# Autodesk Inventor assembly: CNC-FullAssembly
(part 3 of 3)
- Mate:441: CNC-014-ZAxisSubMount1:1 ↔ 90327A125-M5x10mm-LowProfileSCS:17
- Mate:442: CNC-014-ZAxisSubMount1:1 ↔ 90327A125-M5x10mm-LowProfileSCS:18
- Flush:214: 90327A125-M5x10mm-LowProfileSCS:17 ↔ 90327A125-M5x10mm-LowProfileSCS:18
- Flush:215: 90327A125-M5x10mm-LowProfileSCS:13 ↔ 90327A125-M5x10mm-LowProfileSCS:17
- Mate:443: BF12-BallScrewStabilizer2:1 ↔ 91290A195-M5x35mm:2
- Mate:444: BF12-BallScrewStabilizer2:1 ↔ 91290A195-M5x35mm:4
- Mate:445: BF12-BallScrewStabilizer2:1 ↔ 91290A195-M5x35mm:1
- Mate:446: BF12-BallScrewStabilizer2:1 ↔ 91290A195-M5x35mm:3
- Mate:447: BF12-BallScrewStabilizer2:1 ↔ 91290A195-M5x35mm:3
- Flush:216: 91290A195-M5x35mm:2 ↔ 91290A195-M5x35mm:3
- Flush:217: 91290A195-M5x35mm:2 ↔ 91290A195-M5x35mm:4
- Flush:218: 91290A195-M5x35mm:1 ↔ 91290A195-M5x35mm:4
- Mate:448: 91290A195-M5x35mm:2 ↔ 90576A104-M5-NylockNut:9
- Mate:449: 91290A195-M5x35mm:3 ↔ 90576A104-M5-NylockNut:10
- Mate:450: 91290A195-M5x35mm:4 ↔ 90576A104-M5-NylockNut:11
- Mate:451: 91290A195-M5x35mm:1 ↔ 90576A104-M5-NylockNut:12
- Mate:452: CNC-001-StructureGusset2:1 ↔ 90576A104-M5-NylockNut:9
- Flush:219: 90576A104-M5-NylockNut:9 ↔ 90576A104-M5-NylockNut:10
- Flush:220: 90576A104-M5-NylockNut:10 ↔ 90576A104-M5-NylockNut:12
- Flush:221: 90576A104-M5-NylockNut:11 ↔ 90576A104-M5-NylockNut:12
- Mate:453: RouterSpindle-65mm:1 ↔ CNC-015-65mmSpindleMount:1
- Mate:454: RouterSpindle-65mm:1 ↔ CNC-015-65mmSpindleMount:1
- Mate:455: HGR20R-LinearRail200mm:2 ↔ 20x20x250mm_Extrusion:1
- Flush:222: HGR20R-LinearRail200mm:2 ↔ 20x20x250mm_Extrusion:1
- Flush:223: HGR20R-LinearRail200mm:2 ↔ 20x20x250mm_Extrusion:1
- Mate:456: HGR20R-LinearRail200mm:1 ↔ 20x20x250mm_Extrusion:2
- Flush:224: HGR20R-LinearRail200mm:1 ↔ 20x20x250mm_Extrusion:2
- Flush:225: 20x20x250mm_Extrusion:1 ↔ 20x20x250mm_Extrusion:2
- Mate:457: HGR20R-LinearRail200mm:2 ↔ 91290A231-M5x15mm:100
- Mate:458: HGR20R-LinearRail200mm:2 ↔ 91290A231-M5x15mm:100
- Mate:459: HGR20R-LinearRail200mm:1 ↔ 91290A231-M5x15mm:101
- Mate:460: HGR20R-LinearRail200mm:1 ↔ 91290A231-M5x15mm:102
- Mate:461: HGR20R-LinearRail200mm:1 ↔ 91290A231-M5x15mm:103
- Mate:462: HGR20R-LinearRail200mm:2 ↔ 91290A231-M5x15mm:104
- Mate:463: HGR20R-LinearRail200mm:2 ↔ 91290A231-M5x15mm:105
- Flush:226: 91290A231-M5x15mm:104 ↔ 91290A231-M5x15mm:105
- Flush:227: 91290A231-M5x15mm:100 ↔ 91290A231-M5x15mm:104
- Flush:228: 91290A231-M5x15mm:100 ↔ 91290A231-M5x15mm:101
- Flush:229: 91290A231-M5x15mm:101 ↔ 91290A231-M5x15mm:102
- Flush:230: 91290A231-M5x15mm:102 ↔ 91290A231-M5x15mm:103
- Mate:464: HGR20R-LinearRail200mm:1 ↔ 91290A231-M5x15mm:106
- Mate:465: HGR20R-LinearRail200mm:2 ↔ 91290A231-M5x15mm:107
- Flush:231: 91290A231-M5x15mm:100 ↔ 91290A231-M5x15mm:107
- Flush:232: 91290A231-M5x15mm:100 ↔ 91290A231-M5x15mm:106
- Angle:23 (0 deg): CNC-015-65mmSpindleMount:1 ↔ 20x20x250mm_Extrusion:1
- Mate:466: CNC-014-ZAxisSubMount1:1 ↔ 90327A125-M5x10mm-LowProfileSCS:19
- Mate:467: CNC-014-ZAxisSubMount1:1 ↔ 90327A125-M5x10mm-LowProfileSCS:20
- Flush:233: 90327A125-M5x10mm-LowProfileSCS:19 ↔ 90327A125-M5x10mm-LowProfileSCS:20
- Flush:234: 90327A125-M5x10mm-LowProfileSCS:16 ↔ 90327A125-M5x10mm-LowProfileSCS:19
- Mate:468: BF12-BallScrewStabilizer2:3 ↔ CNC-016-SpindleMountPlate:1
- Mate:469: BF12-BallScrewStabilizer2:3 ↔ CNC-016-SpindleMountPlate:1
- Mate:470: 20x20x250mm_Extrusion:2 ↔ CNC-016-SpindleMountPlate:1
- Mate:471: CNC-016-SpindleMountPlate:1 ↔ 90576A104-M5-NylockNut:13
- Mate:472: CNC-016-SpindleMountPlate:1 ↔ 90576A104-M5-NylockNut:13
- Mate:473: CNC-016-SpindleMountPlate:1 ↔ 90576A104-M5-NylockNut:14
- Flush:235: 90576A104-M5-NylockNut:13 ↔ 90576A104-M5-NylockNut:14
- Mate:474: CNC-016-SpindleMountPlate:1 ↔ 90576A104-M5-NylockNut:15
- Mate:475: CNC-016-SpindleMountPlate:1 ↔ 90576A104-M5-NylockNut:16
- Flush:236: 90576A104-M5-NylockNut:15 ↔ 90576A104-M5-NylockNut:16
- Flush:237: 90576A104-M5-NylockNut:13 ↔ 90576A104-M5-NylockNut:15
- Mate:476: CNC-015-65mmSpindleMount:1 ↔ 91274A131_M5x20mm:23
- Mate:477: CNC-015-65mmSpindleMount:1 ↔ 91274A131_M5x20mm:24
- Mate:478: CNC-015-65mmSpindleMount:1 ↔ 91274A131_M5x20mm:25
- Mate:479: CNC-015-65mmSpindleMount:1 ↔ 91274A131_M5x20mm:26
- Flush:238: 91274A131_M5x20mm:25 ↔ 91274A131_M5x20mm:26
- Flush:239: 91274A131_M5x20mm:23 ↔ 91274A131_M5x20mm:26
- Flush:240: 91274A131_M5x20mm:23 ↔ 91274A131_M5x20mm:24
- Mate:480: CNC-015-65mmSpindleMount:1 ↔ 91274A131_M5x20mm:23
- Mate:481: CNC-016-SpindleMountPlate:1 ↔ 90327A125-M5x10mm-LowProfileSCS:21
- Mate:482: CNC-016-SpindleMountPlate:1 ↔ 90327A125-M5x10mm-LowProfileSCS:21
- Mate:483: CNC-016-SpindleMountPlate:1 ↔ 90327A125-M5x10mm-LowProfileSCS:22
- Flush:241: 90327A125-M5x10mm-LowProfileSCS:21 ↔ 90327A125-M5x10mm-LowProfileSCS:22
- Mate:484: CNC-016-SpindleMountPlate:1 ↔ 90327A125-M5x10mm-LowProfileSCS:23
- Mate:485: CNC-016-SpindleMountPlate:1 ↔ 90327A125-M5x10mm-LowProfileSCS:24
- Flush:242: 90327A125-M5x10mm-LowProfileSCS:23 ↔ 90327A125-M5x10mm-LowProfileSCS:24
- Flush:243: 90327A125-M5x10mm-LowProfileSCS:22 ↔ 90327A125-M5x10mm-LowProfileSCS:23
- Mate:486: CNC-016-SpindleMountPlate:1 ↔ 90327A125-M5x10mm-LowProfileSCS:26
- Mate:487: CNC-016-SpindleMountPlate:1 ↔ 90327A125-M5x10mm-LowProfileSCS:27
- Mate:488: CNC-016-SpindleMountPlate:1 ↔ 90327A125-M5x10mm-LowProfileSCS:25
- Mate:489: CNC-016-SpindleMountPlate:1 ↔ 90327A125-M5x10mm-LowProfileSCS:28
- Flush:244: 90327A125-M5x10mm-LowProfileSCS:25 ↔ 90327A125-M5x10mm-LowProfileSCS:28
- Flush:245: 90327A125-M5x10mm-LowProfileSCS:27 ↔ 90327A125-M5x10mm-LowProfileSCS:28
- Flush:246: 90327A125-M5x10mm-LowProfileSCS:26 ↔ 90327A125-M5x10mm-LowProfileSCS:27
- Flush:247: 90327A125-M5x10mm-LowProfileSCS:21 ↔ 90327A125-M5x10mm-LowProfileSCS:26
- Mate:490: BK12-BallScrewStabilizer:3 ↔ 92981A790-M5x40mm-ShoulderBolt:5
- Mate:491: BK12-BallScrewStabilizer:3 ↔ 92981A790-M5x40mm-ShoulderBolt:3
- Mate:492: BK12-BallScrewStabilizer:3 ↔ 92981A790-M5x40mm-ShoulderBolt:4
- Mate:493: BK12-BallScrewStabilizer:3 ↔ 92981A790-M5x40mm-ShoulderBolt:6
- Mate:494: BK12-BallScrewStabilizer:3 ↔ 92981A790-M5x40mm-ShoulderBolt:6
- Flush:248: 92981A790-M5x40mm-ShoulderBolt:4 ↔ 92981A790-M5x40mm-ShoulderBolt:6
- Flush:249: 92981A790-M5x40mm-ShoulderBolt:4 ↔ 92981A790-M5x40mm-ShoulderBolt:5
- Flush:250: 92981A790-M5x40mm-ShoulderBolt:3 ↔ 92981A790-M5x40mm-ShoulderBolt:5
- Mate:495: BK12-BallScrewStabilizer:3 ↔ CNC-017-SpindleMountPlate2:1
- Mate:496: BK12-BallScrewStabilizer:3 ↔ CNC-017-SpindleMountPlate2:1
- Mate:497: 20x20x250mm_Extrusion:1 ↔ CNC-017-SpindleMountPlate2:1
- Mate:498: CNC-017-SpindleMountPlate2:1 ↔ 90327A125-M5x10mm-LowProfileSCS:30
- Mate:499: CNC-017-SpindleMountPlate2:1 ↔ 90327A125-M5x10mm-LowProfileSCS:29
- Mate:500: CNC-017-SpindleMountPlate2:1 ↔ 90327A125-M5x10mm-LowProfileSCS:31
- Mate:501: CNC-017-SpindleMountPlate2:1 ↔ 90327A125-M5x10mm-LowProfileSCS:32
- Mate:502: CNC-017-SpindleMountPlate2:1 ↔ 90327A125-M5x10mm-LowProfileSCS:32
- Flush:251: 90327A125-M5x10mm-LowProfileSCS:31 ↔ 90327A125-M5x10mm-LowProfileSCS:32
- Flush:252: 90327A125-M5x10mm-LowProfileSCS:29 ↔ 90327A125-M5x10mm-LowProfileSCS:32
- Flush:253: 90327A125-M5x10mm-LowProfileSCS:29 ↔ 90327A125-M5x10mm-LowProfileSCS:30
- Mate:503: CNC-015-65mmSpindleMount:1 ↔ 91274A134-M5x30mm:5
- Mate:504: CNC-015-65mmSpindleMount:1 ↔ 91274A134-M5x30mm:6
- Mate:505: CNC-015-65mmSpindleMount:1 ↔ 91274A134-M5x30mm:6
- Mate:506: CNC-015-65mmSpindleMount:1 ↔ 91274A134-M5x30mm:5
- Mate:507: 91274A134-M5x30mm:5 ↔ 90576A104-M5-NylockNut:18
- Mate:508: 91274A134-M5x30mm:6 ↔ 90576A104-M5-NylockNut:17
- Mate:509: CNC-015-65mmSpindleMount:1 ↔ 90576A104-M5-NylockNut:17
- Flush:254: 90576A104-M5-NylockNut:17 ↔ 90576A104-M5-NylockNut:18
- Mate:510: BK12-BallScrewStabilizer:3 ↔ CNC-018-ZAxisBallScrewStabilizerShim1:1
- Mate:511: BK12-BallScrewStabilizer:3 ↔ CNC-018-ZAxisBallScrewStabilizerShim1:1
- Mate:512: CNC-017-SpindleMountPlate2:1 ↔ CNC-018-ZAxisBallScrewStabilizerShim1:1
- Mate:513: BF12-BallScrewStabilizer2:3 ↔ CNC-019-ZAxisBallScrewStabilizerShim2:1
- Mate:514: BF12-BallScrewStabilizer2:3 ↔ CNC-019-ZAxisBallScrewStabilizerShim2:1
- Mate:515: CNC-016-SpindleMountPlate:1 ↔ CNC-019-ZAxisBallScrewStabilizerShim2:1
- Mate:516: 20x20x250mm_Extrusion:1 ↔ CNC-020-ZAxisNema23Mount:1
- Mate:517: 20x20x250mm_Extrusion:2 ↔ CNC-020-ZAxisNema23Mount:1
- Mate:518: 20x20x250mm_Extrusion:1 ↔ CNC-020-ZAxisNema23Mount:1
- Flush:255: 20x40x500mm-Extrusion:2 ↔ 20x40x350mm-ExtrusionNoHoles:1
- Mate:520 (44 mm): 20x40x500mm-Extrusion:1 ↔ 20x40x350mm-ExtrusionNoHoles:1
- Mate:521: CNC-020-ZAxisNema23Mount:1 ↔ 91274A131_M5x20mm:29
- Mate:522: CNC-020-ZAxisNema23Mount:1 ↔ 91274A131_M5x20mm:30
- Mate:523: CNC-020-ZAxisNema23Mount:1 ↔ 91274A131_M5x20mm:30
- Flush:256: 91274A131_M5x20mm:29 ↔ 91274A131_M5x20mm:30
- Mate:524: Nema23-StepperMotor:3 ↔ 91274A131_M5x20mm:32
- Mate:525: Nema23-StepperMotor:3 ↔ 91274A131_M5x20mm:31
- Mate:526: Nema23-StepperMotor:3 ↔ 91274A131_M5x20mm:33
- Mate:527: Nema23-StepperMotor:3 ↔ 91274A131_M5x20mm:34
- Mate:528: Nema23-StepperMotor:3 ↔ 91274A131_M5x20mm:34
- Flush:257: 91274A131_M5x20mm:31 ↔ 91274A131_M5x20mm:34
- Flush:258: 91274A131_M5x20mm:31 ↔ 91274A131_M5x20mm:33
- Flush:259: 91274A131_M5x20mm:32 ↔ 91274A131_M5x20mm:33
- Mate:529: CNC-007-XAxisBallScrewMount:1 ↔ 91274A134-M5x30mm:10
- Mate:530: CNC-007-XAxisBallScrewMount:1 ↔ 91274A134-M5x30mm:9
- Mate:531: CNC-007-XAxisBallScrewMount:1 ↔ 91274A134-M5x30mm:8
- Mate:532: CNC-007-XAxisBallScrewMount:1 ↔ 91274A134-M5x30mm:7
- Mate:533: CNC-007-XAxisBallScrewMount:1 ↔ 91274A134-M5x30mm:7
- Flush:260: 91274A134-M5x30mm:7 ↔ 91274A134-M5x30mm:9
- Flush:261: 91274A134-M5x30mm:9 ↔ 91274A134-M5x30mm:10
- Flush:262: 91274A134-M5x30mm:8 ↔ 91274A134-M5x30mm:10
- Mate:534: 91274A131_M5x20mm:31 ↔ 90576A104-M5-NylockNut:20
- Mate:535: 91274A131_M5x20mm:32 ↔ 90576A104-M5-NylockNut:19
- Mate:536: 91274A131_M5x20mm:34 ↔ 90576A104-M5-NylockNut:22
- Mate:537: 91274A131_M5x20mm:33 ↔ 90576A104-M5-NylockNut:21
- Mate:538: CNC-020-ZAxisNema23Mount:1 ↔ 90576A104-M5-NylockNut:21
- Flush:263: 90576A104-M5-NylockNut:19 ↔ 90576A104-M5-NylockNut:21
- Flush:264: 90576A104-M5-NylockNut:19 ↔ 90576A104-M5-NylockNut:20
- Flush:265: 90576A104-M5-NylockNut:20 ↔ 90576A104-M5-NylockNut:22
- Mate:539: 91274A134-M5x30mm:7 ↔ 90576A104-M5-NylockNut:24
- Mate:540: 91274A134-M5x30mm:9 ↔ 90576A104-M5-NylockNut:26
- Mate:541: 91274A134-M5x30mm:10 ↔ 90576A104-M5-NylockNut:25
- Mate:542: 91274A134-M5x30mm:8 ↔ 90576A104-M5-NylockNut:23
- Mate:543: BF12-BallScrewStabilizer2:2 ↔ 90576A104-M5-NylockNut:23
- Flush:266: 90576A104-M5-NylockNut:23 ↔ 90576A104-M5-NylockNut:25
- Flush:267: 90576A104-M5-NylockNut:23 ↔ 90576A104-M5-NylockNut:24
- Flush:268: 90576A104-M5-NylockNut:24 ↔ 90576A104-M5-NylockNut:26
- Angle:24 (0 deg): 20x20x250mm_Extrusion:1 ↔ 3103-0001-0002-GobildaLimitSwitch:3
- Angle:25 (0 deg): 20x20x250mm_Extrusion:1 ↔ 3103-0001-0002-GobildaLimitSwitch:3
- Mate:544: 3103-0001-0002-GobildaLimitSwitch:3 ↔ CNC-021-ZAxisLimitSwitchMount:1
- Mate:545: 3103-0001-0002-GobildaLimitSwitch:3 ↔ CNC-021-ZAxisLimitSwitchMount:1
- Tangent:12: 20x20x250mm_Extrusion:1 ↔ CNC-021-ZAxisLimitSwitchMount:1
- Mate:546: 3103-0001-0002-GobildaLimitSwitch:3 ↔ CNC-021-ZAxisLimitSwitchMount:1
- Mate:547: 3103-0001-0002-GobildaLimitSwitch:3 ↔ 90480A003-#2-HexNut:6
- Mate:548: 3103-0001-0002-GobildaLimitSwitch:3 ↔ 90480A003-#2-HexNut:5
- Mate:549: 3103-0001-0002-GobildaLimitSwitch:3 ↔ 90480A003-#2-HexNut:6
- Flush:270: 90480A003-#2-HexNut:5 ↔ 90480A003-#2-HexNut:6
- Mate:550: 90480A003-#2-HexNut:5 ↔ 90128A046-#2-.375in:5
- Mate:551: 90480A003-#2-HexNut:6 ↔ 90128A046-#2-.375in:6
- Flush:271: 90128A046-#2-.375in:5 ↔ 90128A046-#2-.375in:6
- Mate:552: CNC-021-ZAxisLimitSwitchMount:1 ↔ 90128A046-#2-.375in:6
- Mate:553: CNC-021-ZAxisLimitSwitchMount:1 ↔ 90327A125-M5x10mm-LowProfileSCS:33
- Mate:554: CNC-021-ZAxisLimitSwitchMount:1 ↔ 90327A125-M5x10mm-LowProfileSCS:34
- Mate:555: CNC-021-ZAxisLimitSwitchMount:1 ↔ 90327A125-M5x10mm-LowProfileSCS:34
- Flush:272: 90327A125-M5x10mm-LowProfileSCS:33 ↔ 90327A125-M5x10mm-LowProfileSCS:34
- Mate:556: 20x20x250mm_Extrusion:1 ↔ CNC-021-ZAxisLimitSwitchMount:1
- Flush:273 (4.7625 mm): 20x20x250mm_Extrusion:1 ↔ CNC-021-ZAxisLimitSwitchMount:1
- Mate:557: BK12-BallScrewStabilizer:2 ↔ CNC-022-XAxisBallScrewStabilizerMount:1
- Mate:558: BK12-BallScrewStabilizer:2 ↔ CNC-022-XAxisBallScrewStabilizerMount:1
- Mate:559: BK12-BallScrewStabilizer:2 ↔ CNC-022-XAxisBallScrewStabilizerMount:1
- Mate:560: CNC-022-XAxisBallScrewStabilizerMount:1 ↔ 91290A195-M5x35mm:5
- Mate:561: CNC-022-XAxisBallScrewStabilizerMount:1 ↔ 91290A195-M5x35mm:6
- Mate:562: CNC-022-XAxisBallScrewStabilizerMount:1 ↔ 91290A195-M5x35mm:6
- Flush:274: 91290A195-M5x35mm:5 ↔ 91290A195-M5x35mm:6
- Mate:563: CNC-022-XAxisBallScrewStabilizerMount:1 ↔ 91290A195-M5x35mm:8
- Flush:275: 91290A195-M5x35mm:5 ↔ 91290A195-M5x35mm:8
- Mate:564: CNC-022-XAxisBallScrewStabilizerMount:1 ↔ 91290A195-M5x35mm:7
- Flush:276: 91290A195-M5x35mm:6 ↔ 91290A195-M5x35mm:7
- Mate:565: CNC-022-XAxisBallScrewStabilizerMount:1 ↔ 91274A125-M5x8mm:41
- Mate:566: CNC-022-XAxisBallScrewStabilizerMount:1 ↔ 91274A125-M5x8mm:42
- Mate:567: CNC-022-XAxisBallScrewStabilizerMount:1 ↔ 91274A125-M5x8mm:42
- Flush:277: 91274A125-M5x8mm:41 ↔ 91274A125-M5x8mm:42
- Mate:568: 91290A195-M5x35mm:6 ↔ 90576A104-M5-NylockNut:27
- Mate:569: 91290A195-M5x35mm:7 ↔ 90576A104-M5-NylockNut:28
- Mate:570: BK12-BallScrewStabilizer:2 ↔ 90576A104-M5-NylockNut:28
- Flush:278: 90576A104-M5-NylockNut:27 ↔ 90576A104-M5-NylockNut:28
- Mate:571: 91290A195-M5x35mm:5 ↔ 90576A104-M5-NylockNut:29
- Flush:279: 90576A104-M5-NylockNut:27 ↔ 90576A104-M5-NylockNut:29
- Mate:572: 91290A195-M5x35mm:8 ↔ 90576A104-M5-NylockNut:30
- Flush:280: 90576A104-M5-NylockNut:29 ↔ 90576A104-M5-NylockNut:30
- Mate:573: BK12-BallScrewStabilizer:1 ↔ CNC-023-YAxisBallScrewStabilizerMount:1
- Mate:574: BK12-BallScrewStabilizer:1 ↔ CNC-023-YAxisBallScrewStabilizerMount:1
- Mate:575: BK12-BallScrewStabilizer:1 ↔ CNC-023-YAxisBallScrewStabilizerMount:1
- Mate:576: CNC-023-YAxisBallScrewStabilizerMount:1 ↔ 91290A231-M5x15mm:108
- Mate:577: CNC-023-YAxisBallScrewStabilizerMount:1 ↔ 91290A231-M5x15mm:108
- Mate:578: CNC-023-YAxisBallScrewStabilizerMount:1 ↔ 91290A231-M5x15mm:110
- Flush:281: 91290A231-M5x15mm:108 ↔ 91290A231-M5x15mm:110
- Mate:579: CNC-023-YAxisBallScrewStabilizerMount:1 ↔ 91290A231-M5x15mm:109
- Mate:580: CNC-023-YAxisBallScrewStabilizerMount:1 ↔ 91290A231-M5x15mm:111
- Mate:581: CNC-023-YAxisBallScrewStabilizerMount:1 ↔ 91290A231-M5x15mm:111
- Flush:282: 91290A231-M5x15mm:109 ↔ 91290A231-M5x15mm:111
- Mate:582: BK12-BallScrewStabilizer:1 ↔ 91292A195-M5x45mm:10
- Mate:583: BK12-BallScrewStabilizer:1 ↔ 91292A195-M5x45mm:10
- Mate:584: BK12-BallScrewStabilizer:1 ↔ 91292A195-M5x45mm:12
- Flush:283: 91292A195-M5x45mm:10 ↔ 91292A195-M5x45mm:12
- Mate:585: BK12-BallScrewStabilizer:1 ↔ 91292A195-M5x45mm:11
- Flush:284: 91292A195-M5x45mm:10 ↔ 91292A195-M5x45mm:11
- Mate:586: BK12-BallScrewStabilizer:1 ↔ 91292A195-M5x45mm:9
- Flush:285: 91292A195-M5x45mm:9 ↔ 91292A195-M5x45mm:12
- Mate:587: 91292A195-M5x45mm:12 ↔ 90576A104-M5-NylockNut:31
- Mate:588: CNC-023-YAxisBallScrewStabilizerMount:1 ↔ 90576A104-M5-NylockNut:31
- Mate:589: 91292A195-M5x45mm:9 ↔ 90576A104-M5-NylockNut:33
- Flush:286: 90576A104-M5-NylockNut:31 ↔ 90576A104-M5-NylockNut:33
- Mate:590: 91292A195-M5x45mm:10 ↔ 90576A104-M5-NylockNut:34
- Flush:287: 90576A104-M5-NylockNut:31 ↔ 90576A104-M5-NylockNut:34
- Mate:591: 91292A195-M5x45mm:11 ↔ 90576A104-M5-NylockNut:32
- Flush:288: 90576A104-M5-NylockNut:32 ↔ 90576A104-M5-NylockNut:34
- Tangent:13: 40x40x500mm-Extrusion:1 ↔ CNC-024-MillFeet:1
- Tangent:14: 40x40x500mm-Extrusion:1 ↔ CNC-024-MillFeet:1
- Flush:289: 40x40x500mm-Extrusion:1 ↔ CNC-024-MillFeet:1
- Mate:592: 40x40x500mm-Extrusion:1 ↔ CNC-024-MillFeet:1
- Flush:290: CNC-024-MillFeet:1 ↔ CNC-024-MillFeet:2
- Mate:593: 40x40x500mm-Extrusion:1 ↔ CNC-024-MillFeet:2
- Flush:291: 40x40x500mm-Extrusion:1 ↔ CNC-024-MillFeet:2
- Angle:26 (0 deg): 40x40x500mm-Extrusion:2 ↔ CNC-024-MillFeet:3
- Tangent:15: 40x40x500mm-Extrusion:2 ↔ CNC-024-MillFeet:3
- Mate:594: 40x40x500mm-Extrusion:2 ↔ CNC-024-MillFeet:3
- Flush:292: 40x40x500mm-Extrusion:2 ↔ CNC-024-MillFeet:3
- Flush:293: CNC-024-MillFeet:3 ↔ CNC-024-MillFeet:4
- Flush:294: CNC-024-MillFeet:3 ↔ CNC-024-MillFeet:4
- Flush:295: CNC-024-MillFeet:2 ↔ CNC-024-MillFeet:4
- Mate:595: CNC-024-MillFeet:4 ↔ 91290A231-M5x15mm:114
- Mate:596: CNC-024-MillFeet:3 ↔ 91290A231-M5x15mm:115
- Mate:597: CNC-024-MillFeet:1 ↔ 91290A231-M5x15mm:113
- Mate:598: CNC-024-MillFeet:2 ↔ 91290A231-M5x15mm:112
- Mate:599: CNC-024-MillFeet:2 ↔ 91290A231-M5x15mm:112
- Flush:296: 91290A231-M5x15mm:113 ↔ 91290A231-M5x15mm:112
- Flush:297: 91290A231-M5x15mm:115 ↔ 91290A231-M5x15mm:113
- Flush:298: 91290A231-M5x15mm:114 ↔ 91290A231-M5x15mm:115
- Angle:27 (0 deg): 40x40x500mm-Extrusion:2 ↔ 10x15-CableCarrierYAxis-2924-1015-1000:1
- Angle:28 (0 deg): 40x40x500mm-Extrusion:2 ↔ 10x15-CableCarrierYAxis-2924-1015-1000:1
- Mate:600 (6.35 mm): 40x40x500mm-Extrusion:2 ↔ 10x15-CableCarrierYAxis-2924-1015-1000:1
- Flush:299 (15 mm): 40x40x500mm-Extrusion:2 ↔ 10x15-CableCarrierYAxis-2924-1015-1000:1
- Mate:601: 20x40x500mm-Extrusion2:2 ↔ CNC-022-XAxisBallScrewStabilizerMount:1
- Mate:602: CNC-006-XAxisMount2:1 ↔ CNC-025-YAxisCableCarrierMount:1
- Mate:603: CNC-006-XAxisMount2:1 ↔ CNC-025-YAxisCableCarrierMount:1
- Mate:604: CNC-006-XAxisMount2:1 ↔ CNC-025-YAxisCableCarrierMount:1
- Mate:605: CNC-025-YAxisCableCarrierMount:1 ↔ 91274A117-M4x10mm:1
- Mate:606: CNC-025-YAxisCableCarrierMount:1 ↔ 91274A117-M4x10mm:1
- Mate:607: CNC-025-YAxisCableCarrierMount:1 ↔ 91274A117-M4x10mm:2
- Flush:300: 91274A117-M4x10mm:1 ↔ 91274A117-M4x10mm:2
- Angle:29 (0 deg): 40x40x500mm-Extrusion:2 ↔ CNC-026-CableCarrierTrack:1
- Mate:608: 40x40x500mm-Extrusion:2 ↔ CNC-026-CableCarrierTrack:1
- Tangent:16: 40x40x500mm-Extrusion:2 ↔ CNC-026-CableCarrierTrack:1
- Flush:302: CNC-026-CableCarrierTrack:1 ↔ CNC-026-CableCarrierTrack:2
- Flush:303: CNC-026-CableCarrierTrack:1 ↔ CNC-026-CableCarrierTrack:2
- Flush:305: CNC-026-CableCarrierTrack:2 ↔ CNC-026-CableCarrierTrack:3
- Flush:306: CNC-026-CableCarrierTrack:1 ↔ CNC-026-CableCarrierTrack:3
- Mate:609: CNC-026-CableCarrierTrack:3 ↔ 91274A125-M5x8mm:46
- Mate:610: CNC-026-CableCarrierTrack:3 ↔ 91274A125-M5x8mm:48
- Mate:611: CNC-026-CableCarrierTrack:1 ↔ 91274A125-M5x8mm:47
- Mate:612: CNC-026-CableCarrierTrack:1 ↔ 91274A125-M5x8mm:44
- Mate:613: CNC-026-CableCarrierTrack:2 ↔ 91274A125-M5x8mm:43
- Mate:614: CNC-026-CableCarrierTrack:2 ↔ 91274A125-M5x8mm:45
- Mate:615: CNC-026-CableCarrierTrack:2 ↔ 91274A125-M5x8mm:45
- Flush:308: 91274A125-M5x8mm:43 ↔ 91274A125-M5x8mm:45
- Flush:309: 91274A125-M5x8mm:43 ↔ 91274A125-M5x8mm:46
- Flush:310: 91274A125-M5x8mm:46 ↔ 91274A125-M5x8mm:48
- Flush:311: 91274A125-M5x8mm:44 ↔ 91274A125-M5x8mm:46
- Flush:312: 91274A125-M5x8mm:44 ↔ 91274A125-M5x8mm:47
- Mate:616: CNC-006-XAxisMount2:1 ↔ CNC-027-XAxisWireDuct:1
- Mate:618: CNC-006-XAxisMount2:1 ↔ CNC-027-XAxisWireDuct:1
- Mate:619: CNC-006-XAxisMount2:1 ↔ 91274A117-M4x10mm:3
- Mate:620: CNC-027-XAxisWireDuct:1 ↔ 91274A117-M4x10mm:3
- Mate:621: CNC-027-XAxisWireDuct:1 ↔ 91274A117-M4x10mm:4
- Flush:313: 91274A117-M4x10mm:3 ↔ 91274A117-M4x10mm:4
- Angle:30 (0 deg): CNC-006-XAxisMount2:1 ↔ CNC-027-XAxisWireDuct:1
- Flush:314: CNC-003-StructureGusset3:2 ↔ CNC-028-WireTrack1:1
- Flush:315: CNC-003-StructureGusset3:2 ↔ CNC-028-WireTrack1:1
- Mate:622: CNC-028-WireTrack1:1 ↔ 91290A231-M5x15mm:128
- Mate:623: CNC-028-WireTrack1:1 ↔ 91290A231-M5x15mm:128
- Mate:624: 40x40x500mm-Extrusion:1 ↔ CNC-012-YAxisLimitSwitchMount:2
- Flush:316 (0.4587 mm): 40x40x500mm-Extrusion:1 ↔ CNC-012-YAxisLimitSwitchMount:2
- Tangent:17: 40x40x500mm-Extrusion:1 ↔ CNC-012-YAxisLimitSwitchMount:2
- Mate:625: CNC-012-YAxisLimitSwitchMount:2 ↔ 3103-0001-0002-GobildaLimitSwitch:4
- Mate:626: CNC-012-YAxisLimitSwitchMount:2 ↔ 3103-0001-0002-GobildaLimitSwitch:4
- Mate:627: CNC-012-YAxisLimitSwitchMount:2 ↔ 90327A125-M5x10mm-LowProfileSCS:35
- Mate:628: CNC-012-YAxisLimitSwitchMount:2 ↔ 90327A125-M5x10mm-LowProfileSCS:36
- Mate:629: CNC-012-YAxisLimitSwitchMount:2 ↔ 90327A125-M5x10mm-LowProfileSCS:36
- Flush:317: 90327A125-M5x10mm-LowProfileSCS:35 ↔ 90327A125-M5x10mm-LowProfileSCS:36
- Mate:630: 3103-0001-0002-GobildaLimitSwitch:4 ↔ 90128A046-#2-.375in:7
- Mate:631: 3103-0001-0002-GobildaLimitSwitch:4 ↔ 90128A046-#2-.375in:8
- Flush:318: 90128A046-#2-.375in:7 ↔ 90128A046-#2-.375in:8
- Mate:632: 3103-0001-0002-GobildaLimitSwitch:4 ↔ 90128A046-#2-.375in:7
- Mate:633: CNC-012-YAxisLimitSwitchMount:2 ↔ 3103-0001-0002-GobildaLimitSwitch:4
- Mate:634: 90128A046-#2-.375in:7 ↔ 90480A003-#2-HexNut:8
- Mate:635: 90128A046-#2-.375in:8 ↔ 90480A003-#2-HexNut:7
- Flush:319: 90480A003-#2-HexNut:7 ↔ 90480A003-#2-HexNut:8
- Angle:31 (0 deg): CNC-012-YAxisLimitSwitchMount:2 ↔ 90480A003-#2-HexNut:8
- Mate:636: CNC-012-YAxisLimitSwitchMount:2 ↔ 90480A003-#2-HexNut:8
- Symmetry:1: CNC-003-StructureGusset3:1 ↔ CNC-003-StructureGusset3:2
- Mate:637: CNC-028-WireTrack1_MIR:1 ↔ 91290A231-M5x15mm:131
- Mate:638: CNC-028-WireTrack1_MIR:1 ↔ 91290A231-M5x15mm:132
- Mate:639: CNC-028-WireTrack1_MIR:1 ↔ 91290A231-M5x15mm:133
- Mate:640: CNC-003-StructureGusset3:1 ↔ CNC-028-WireTrack1_MIR:1
- Mate:641: CNC-003-StructureGusset3:1 ↔ CNC-028-WireTrack1_MIR:1
- Mate:642: CNC-003-StructureGusset3:1 ↔ CNC-028-WireTrack1_MIR:1
- Mate:643: CNC-028-WireTrack1_MIR:1 ↔ 91290A231-M5x15mm:133
- Flush:320: 91290A231-M5x15mm:132 ↔ 91290A231-M5x15mm:133
- Flush:321: 91290A231-M5x15mm:131 ↔ 91290A231-M5x15mm:132
- Mate:644: CNC-006-XAxisMount2:1 ↔ 10x15-CarbleCarrierXAxis-2924-1015-1000:1
- Angle:32 (0 deg): 20x20x500mm_Extrusion:3 ↔ 10x15-CarbleCarrierXAxis-2924-1015-1000:1
- Mate:645: CNC-006-XAxisMount2:1 ↔ 10x15-CarbleCarrierXAxis-2924-1015-1000:1
- Mate:646: 10x15-CarbleCarrierXAxis-2924-1015-1000:1 ↔ 94500A264-M3-12mm-ButtonHead:1
- Mate:647: 10x15-CarbleCarrierXAxis-2924-1015-1000:1 ↔ 94500A264-M3-12mm-ButtonHead:1
- Mate:648: CNC-025-YAxisCableCarrierMount:1 ↔ 94500A264-M3-12mm-ButtonHead:3
- Mate:649: CNC-025-YAxisCableCarrierMount:1 ↔ 94500A264-M3-12mm-ButtonHead:3
- Mate:650: CNC-025-YAxisCableCarrierMount:1 ↔ 94500A264-M3-12mm-ButtonHead:2
- Mate:651: CNC-025-YAxisCableCarrierMount:1 ↔ 94500A264-M3-12mm-ButtonHead:2
- Mate:652: 94500A264-M3-12mm-ButtonHead:1 ↔ 90576A102-M3-NylockNut:1
- Mate:653: CNC-006-XAxisMount2:1 ↔ 90576A102-M3-NylockNut:1
- Mate:654: 94500A264-M3-12mm-ButtonHead:2 ↔ 90576A102-M3-NylockNut:3
- Mate:655: 94500A264-M3-12mm-ButtonHead:3 ↔ 90576A102-M3-NylockNut:2
- Mate:656: 10x15-CableCarrierYAxis-2924-1015-1000:1 ↔ 90576A102-M3-NylockNut:2
- Flush:322: 90576A102-M3-NylockNut:2 ↔ 90576A102-M3-NylockNut:3
- Mate:657: 10x15-CarbleCarrierXAxis-2924-1015-1000:1 ↔ CNC-030-XAxisCableCarrierMount:1
- Mate:658: 20x40x500mm-Extrusion2:1 ↔ CNC-030-XAxisCableCarrierMount:1
- Mate:659: 10x15-CarbleCarrierXAxis-2924-1015-1000:1 ↔ CNC-030-XAxisCableCarrierMount:1
- Mate:660: CNC-030-XAxisCableCarrierMount:1 ↔ 90327A125-M5x10mm-LowProfileSCS:37
- Mate:661: CNC-030-XAxisCableCarrierMount:1 ↔ 90327A125-M5x10mm-LowProfileSCS:37
- Mate:662: CNC-030-XAxisCableCarrierMount:1 ↔ 94500A264-M3-12mm-ButtonHead:4
- Mate:663: CNC-030-XAxisCableCarrierMount:1 ↔ 94500A264-M3-12mm-ButtonHead:5
- Mate:664: 10x15-CarbleCarrierXAxis-2924-1015-1000:1 ↔ 94500A264-M3-12mm-ButtonHead:4
- Flush:323: 94500A264-M3-12mm-ButtonHead:4 ↔ 94500A264-M3-12mm-ButtonHead:5
- Mate:665: 94500A264-M3-12mm-ButtonHead:4 ↔ 90576A102-M3-NylockNut:4
- Mate:666: CNC-030-XAxisCableCarrierMount:1 ↔ 90576A102-M3-NylockNut:4
- Mate:667: 94500A264-M3-12mm-ButtonHead:5 ↔ 90576A102-M3-NylockNut:5
- Flush:324: 90576A102-M3-NylockNut:4 ↔ 90576A102-M3-NylockNut:5
- Mate:668 (-25.4 mm): 20x40x500mm-Extrusion2:1 ↔ CNC-030-XAxisCableCarrierMount:1
- Flush:325: 91274A125-M5x8mm:32 ↔ 91274A125-M5x8mm:40
- Mate:669 (20 mm): 20x40x500mm-Extrusion:1 ↔ 20x40x350mm-ExtrusionNoHoles:1
- Mate:671: 20x40x350mm-ExtrusionNoHoles:1 ↔ CNC-031-BackCover1:1
- Mate:672: 20x40x500mm-Extrusion:1 ↔ CNC-031-BackCover1:1
- Mate:673: CNC-031-BackCover1:1 ↔ 91290A198-M5-50mm:5
- Mate:674: CNC-031-BackCover1:1 ↔ 91290A198-M5-50mm:5
- Mate:675: CNC-031-BackCover1:1 ↔ 91290A198-M5-50mm:6
- Flush:326: 91290A198-M5-50mm:5 ↔ 91290A198-M5-50mm:6
- Mate:676: CNC-031-BackCover1_MIR:1 ↔ 91290A198-M5-50mm:8
- Mate:677: CNC-031-BackCover1_MIR:1 ↔ 91290A198-M5-50mm:7
- Flush:327: 91290A198-M5-50mm:7 ↔ 91290A198-M5-50mm:8
- Flush:328: 91290A198-M5-50mm:5 ↔ 91290A198-M5-50mm:8
- Mate:678: 20x40x500mm-Extrusion:1 ↔ 91290A198-M5-50mm:5
- Mate:679: 20x40x500mm-Extrusion:2 ↔ CNC-031-BackCover1_MIR:1
- Mate:680: 20x40x500mm-Extrusion:2 ↔ 91290A198-M5-50mm:7
- Mate:681: 20x40x500mm-Extrusion:2 ↔ CNC-031-BackCover1_MIR:1
- Mate:682: CNC-031-BackCover1_MIR2:1 ↔ 91290A198-M5-50mm:9
- Mate:683: CNC-031-BackCover1_MIR2:1 ↔ 91290A198-M5-50mm:10
- Mate:684: CNC-031-BackCover1_MIR2:1 ↔ 91290A198-M5-50mm:10
- Flush:329: 91290A198-M5-50mm:9 ↔ 91290A198-M5-50mm:10
- Mate:685: 20x40x500mm-Extrusion:1 ↔ CNC-031-BackCover1_MIR2:1
- Mate:686: 20x40x500mm-Extrusion:1 ↔ CNC-031-BackCover1_MIR2:1
- Mate:687: 20x40x500mm-Extrusion:1 ↔ CNC-031-BackCover1_MIR2:1
- Mate:688: CNC-031-BackCover1_MIR_MIR3:1 ↔ 91290A198-M5-50mm:11
- Mate:689: CNC-031-BackCover1_MIR_MIR3:1 ↔ 91290A198-M5-50mm:12
- Flush:330: 91290A198-M5-50mm:11 ↔ 91290A198-M5-50mm:12
- Flush:331: 91290A198-M5-50mm:10 ↔ 91290A198-M5-50mm:11
- Mate:690: CNC-031-BackCover1:1 ↔ 91274A125-M5x8mm:49
- Mate:691: CNC-031-BackCover1_MIR2:1 ↔ 91274A125-M5x8mm:50
- Flush:332: 91274A125-M5x8mm:49 ↔ 91274A125-M5x8mm:50
- Flush:333: 91290A198-M5-50mm:6 ↔ 91274A125-M5x8mm:49
